# Autodesk Inventor assembly: Elevator MK2
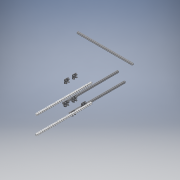
[picture p0: Inventor's stored thumbnail of the model, 180x180]
Saved by Autodesk Inventor 2019.4 (Build 234330000, 330)
## iProperties
Created: 2020-01-23
Part Number: Elevator MK2
Document SubType Name: Assembly
Designer: Mark
Mass: 647.084 g
Surface Area: 2312.45 cm^2
Volume: 239.661 cm^3
Density: 2.7 g/cm^3
Author: Mark
## Documents named in this file (5)
- C:\Users\Mark\Desktop\7738 Helion Engineering\7738-2020\Elevator MK2\Elevator MK2.iam
- C:\Users\Mark\Desktop\7738 Helion Engineering\7738-2020\Spinny disk assembly\Aluminium extrusion profile 2020.ipt
- C:\Users\Mark\Desktop\7738 Helion Engineering\7738-2020\Elevator MK2\Mini V Gantry Kit.ipt
- C:\Users\Mark\Desktop\7738 Helion Engineering\7738-2020\Elevator MK2\Second Stage  Extrusion.ipt
- C:\Users\Mark\Desktop\7738 Helion Engineering\7738-2020\Elevator MK2\Final Stage.ipt
## Components (13 placed, 4 different names)
1. Aluminium extrusion profile 2020:1 — Flush:1, Flush:2, Mate:1
2. Aluminium extrusion profile 2020:2 — Flush:1, Flush:2, Mate:1
3. Mini V Gantry Kit:1 — Mate:12, Mate:13, Mate:14
4. Mini V Gantry Kit:2
5. Mini V Gantry Kit:3 — Mate:18
6. Mini V Gantry Kit:4 — Mate:15, Mate:16, Mate:17
7. Second Stage  Extrusion:1 — Mate:12, Mate:13, Mate:14, Mate:15, Mate:16, Mate:17
8. Second Stage  Extrusion:2 — Mate:18
9. Final Stage:1
10. Mini V Gantry Kit:5
11. Mini V Gantry Kit:6
12. Mini V Gantry Kit:7
13. Mini V Gantry Kit:8
## Relationships (17: Mate 9, Flush 8)
- Flush:1: Aluminium extrusion profile 2020:1 ↔ Aluminium extrusion profile 2020:2
- Flush:2: Aluminium extrusion profile 2020:1 ↔ Aluminium extrusion profile 2020:2
- Mate:1 (200 mm): Aluminium extrusion profile 2020:1 ↔ Aluminium extrusion profile 2020:2
- [Flush]: Mini V Gantry Kit:5 ↔ Mini V Gantry Kit:8
- [Flush]: Mini V Gantry Kit:5 ↔ Mini V Gantry Kit:8
- [Flush]: Mini V Gantry Kit:6 ↔ Mini V Gantry Kit:7
- [Flush]: Mini V Gantry Kit:6 ↔ Mini V Gantry Kit:7
- [Flush]: Mini V Gantry Kit:6 ↔ Mini V Gantry Kit:8
- [Flush]: Mini V Gantry Kit:5 ↔ Mini V Gantry Kit:7
- [Mate] (50 mm): Mini V Gantry Kit:5 ↔ Mini V Gantry Kit:8
- Mate:12: Mini V Gantry Kit:1 ↔ Second Stage  Extrusion:1
- Mate:13: Mini V Gantry Kit:1 ↔ Second Stage  Extrusion:1
- Mate:14: Mini V Gantry Kit:1 ↔ Second Stage  Extrusion:1
- Mate:15: Mini V Gantry Kit:4 ↔ Second Stage  Extrusion:1
- Mate:16: Mini V Gantry Kit:4 ↔ Second Stage  Extrusion:1
- Mate:17: Mini V Gantry Kit:4 ↔ Second Stage  Extrusion:1
- Mate:18: Mini V Gantry Kit:3 ↔ Second Stage  Extrusion:2
## Named parameters: d20_d7 = 0 mm, d21_d12 = 0 mm, d22_d13 = 50 mm, d23_d52 = 0 mm, d24_d53 = 0 mm, d25_d48 = 0 mm, d26_d49 = 0 mm
